# Autodesk Inventor assembly: arduinoWithShield
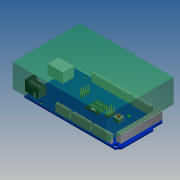
[picture p0: Inventor's stored thumbnail of the model, 180x180]
Saved by Autodesk Inventor 2012 (Build 160160000, 160)
## iProperties
Created: 2012-04-08
Part Number: arduinoWithShield
Document SubType Name: Assembly
Designer: Nathan
Mass: 90.7185 g
Surface Area: 440.61 cm^2
Volume: 204.137 cm^3
Author: Nathan
## Documents named in this file (3)
- C:\Users\Nathan\Desktop\Dropbox\Quadcopter\arduinoWithShield.iam
- C:\Users\Nathan\Desktop\Dropbox\Quadcopter\Imported Components\User Library-Arduino Mega\arduinoMega.iam
- C:\Users\Nathan\Desktop\Dropbox\Quadcopter\shield.ipt
## Components (2 placed, 2 different names)
1. arduinoMega:1 [sub-assembly] — Mate:1, Flush:1, Flush:2
2. shield:1 — Mate:1, Flush:1, Flush:2
## Relationships (3: Flush 2, Mate 1)
- Mate:1 (12.7 mm): arduinoMega:1 ↔ shield:1
- Flush:1: arduinoMega:1 ↔ shield:1
- Flush:2 (-12.7 mm): arduinoMega:1 ↔ shield:1
